# Autodesk Inventor assembly: richInMount
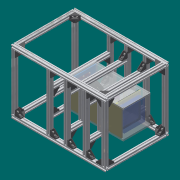
[picture p0: Inventor's stored thumbnail of the model, 180x180]
Saved by Autodesk Inventor 2016 SP1 (Build 200210100, 210)
## iProperties
Created: 2016-02-08
Part Number: richInMount
Document SubType Name: Assembly
Designer: Sawaiz
Author: Sawaiz
## Documents named in this file (5)
- C:\Users\sawaiz\oneDrive\projects\modularRichFrame\richInMount.iam
- C:\Users\sawaiz\oneDrive\projects\modularRichFrame\mainFrame\frame.iam
- C:\Users\sawaiz\OneDrive\projects\modularRICH\modularRICH.iam
- C:\Users\sawaiz\OneDrive\projects\modularRICH\testMount\frame\richHolder.iam
- C:\Users\sawaiz\OneDrive\projects\modularRICH\testMount\frame\richHolderSuppourt.iam
## Components (5 placed, 4 different names)
1. frame:1 [sub-assembly] — Flush:1, Mate:1, Mate:2, Flush:6
2. modularRICH:1 [sub-assembly] — Mate:4, Mate:5, Flush:6, Mate:6
3. richHolder:1 [sub-assembly] — Flush:1, Flush:2, Flush:4, Mate:2, Mate:3, Mate:4, Mate:5
4. richHolder:2 [sub-assembly] — Flush:2, Flush:3, Flush:4, Flush:5, Mate:3
5. richHolderSuppourt:1 [sub-assembly] — Flush:3, Flush:5, Mate:1, Mate:6
## Relationships (12: Flush 6, Mate 6)
- Flush:1: frame:1 ↔ richHolder:1
- Flush:2: richHolder:1 ↔ richHolder:2
- Flush:3: richHolder:2 ↔ richHolderSuppourt:1
- Flush:4: richHolder:1 ↔ richHolder:2
- Flush:5: richHolder:2 ↔ richHolderSuppourt:1
- Mate:1: frame:1 ↔ richHolderSuppourt:1
- Mate:2 (80 mm): frame:1 ↔ richHolder:1
- Mate:3 (80 mm): richHolder:1 ↔ richHolder:2
- Mate:4: modularRICH:1 ↔ richHolder:1
- Mate:5: modularRICH:1 ↔ richHolder:1
- Flush:6: frame:1 ↔ modularRICH:1
- Mate:6: modularRICH:1 ↔ richHolderSuppourt:1
